# Autodesk Inventor assembly: xy ubis mount arm
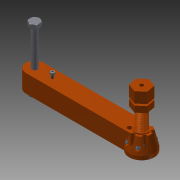
[picture p0: Inventor's stored thumbnail of the model, 180x180]
Saved by Autodesk Inventor 2013 (Build 170138000, 138)
## iProperties
Created: 2013-10-15
Part Number: xy ubis mount arm
Document SubType Name: Assembly
Designer: employee
Author: employee
## Documents named in this file (11)
- C:\Users\employee\Desktop\ConceptFORGE\ConceptFORGE\Wally\INVENTOR\xy ubis mount arm.iam
- C:\Users\employee\Desktop\ConceptFORGE\ConceptFORGE\Wally\INVENTOR\xy ubis mount arm.ipt
- C:\Users\employee\Desktop\ConceptFORGE\ConceptFORGE\Wally\INVENTOR\m3 nut.ipt
- C:\Users\employee\Desktop\ConceptFORGE\ConceptFORGE\Wally\INVENTOR\M3x16.ipt
- C:\Users\employee\Desktop\ConceptFORGE\ConceptFORGE\Wally\INVENTOR\M8 nut.ipt
- C:\Users\employee\Desktop\ConceptFORGE\ConceptFORGE\Wally\INVENTOR\M8x85.ipt
- C:\Users\employee\Desktop\ConceptFORGE\ConceptFORGE\Wally\INVENTOR\bowden nut.ipt
- C:\Users\employee\Desktop\ConceptFORGE\ConceptFORGE\Wally\INVENTOR\lock nut.ipt
- C:\Users\employee\Desktop\ConceptFORGE\ConceptFORGE\Wally\INVENTOR\hub screw.ipt
- C:\Users\employee\Desktop\ConceptFORGE\ConceptFORGE\Wally\INVENTOR\m4 nut.ipt
- C:\Users\employee\Desktop\ConceptFORGE\ConceptFORGE\Wally\INVENTOR\M3x25.ipt
## Components (12 placed, 10 different names)
1. xy ubis mount arm:1 — Angle:1, Angle:2, Insert:7, Insert:8, Insert:9, Mate:2, Insert:13, Insert:14, Insert:15, Insert:16, Insert:17
2. Hex Nut Metric M3 x 0.5:2 — Angle:2, Insert:16
3. Hex Nut Metric M3 x 0.5:3 — Angle:1, Insert:17
4. Forged Socket Head Cap Screw - Metric M3x0.5 x 16:1 — Insert:7
5. Hex Nut Metric M8 x 1.25:1 — Insert:9
6. Hex Bolt - Metric M8 x 1.25 x 70:1 — Insert:8
7. bowden nut:1 — Mate:3, Mate:4
8. lock nut:1 — Mate:2, Mate:3, Mate:5
9. hub screw:1 — Mate:4, Angle:4, Insert:12, Insert:13, Mate:5
10. m4 nut:1 — Angle:4, Insert:12
11. M3x25:1 — Insert:15
12. M3x25:2 — Insert:14
## Relationships (16: Insert 9, Mate 4, Angle 3)
- Angle:1 (0 deg): xy ubis mount arm:1 ↔ Hex Nut Metric M3 x 0.5:3
- Angle:2 (0 deg): xy ubis mount arm:1 ↔ Hex Nut Metric M3 x 0.5:2
- Insert:7 (5 mm): xy ubis mount arm:1 ↔ Forged Socket Head Cap Screw - Metric M3x0.5 x 16:1
- Insert:8 (51.5 mm): xy ubis mount arm:1 ↔ Hex Bolt - Metric M8 x 1.25 x 70:1
- Insert:9: xy ubis mount arm:1 ↔ Hex Nut Metric M8 x 1.25:1
- Mate:2 (26.5 mm): xy ubis mount arm:1 ↔ lock nut:1
- Mate:3: bowden nut:1 ↔ lock nut:1
- Mate:4: bowden nut:1 ↔ hub screw:1
- Angle:4 (0 deg): hub screw:1 ↔ m4 nut:1
- Insert:12: hub screw:1 ↔ m4 nut:1
- Insert:13 (19 mm): xy ubis mount arm:1 ↔ hub screw:1
- Mate:5: lock nut:1 ↔ hub screw:1
- Insert:14: xy ubis mount arm:1 ↔ M3x25:2
- Insert:15: xy ubis mount arm:1 ↔ M3x25:1
- Insert:16: xy ubis mount arm:1 ↔ Hex Nut Metric M3 x 0.5:2
- Insert:17: xy ubis mount arm:1 ↔ Hex Nut Metric M3 x 0.5:3
